# Autodesk Inventor assembly: Space Crush
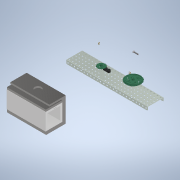
[picture p0: Inventor's stored thumbnail of the model, 180x180]
Saved by Autodesk Inventor 2021 (Build 250183000, 183)
## iProperties
Created: 2021-03-08
Part Number: Space Crush
Document SubType Name: Assembly
Designer: david
Author: david
## Documents named in this file (10)
- C:\Users\david\OneDrive\Documents\Inventor\Space Crush.iam
- C:\Users\david\OneDrive\Documents\Inventor\Inventor_2013_VEX_KOP_-_Imperial\Imperial\Motion\48 Tooth Sprocket.ipt
- C:\Users\david\OneDrive\Documents\Inventor\Inventor_2013_VEX_KOP_-_Imperial\Imperial\Motion\24 Tooth Sprocket.ipt
- C:\Users\david\OneDrive\Documents\Inventor\Inventor_2013_VEX_KOP_-_Imperial\Imperial\Motion\Chain Link.ipt
- C:\Users\david\OneDrive\Documents\Inventor\Inventor_2013_VEX_KOP_-_Imperial\Imperial\Structure\Screw 8-32  x 0.75 inch long.ipt
- C:\Users\david\OneDrive\Documents\Inventor\Inventor_2013_VEX_KOP_-_Imperial\Imperial\Structure\C-Channel 1x5x1x25 Hole.ipt
- C:\Users\david\OneDrive\Documents\Inventor\Inventor_2013_VEX_KOP_-_Imperial\Imperial\Motion\Shaft 2 inch.ipt
- C:\Users\david\OneDrive\Documents\Inventor\Inventor_2013_VEX_KOP_-_Imperial\Imperial\Motion\Bearing Flat.ipt
- C:\Users\david\OneDrive\Documents\Inventor\Clamp for Box Crusher.ipt
- C:\Users\david\OneDrive\Documents\Inventor\Aluminum box 2x2x6 .3 thickness.ipt
## Components (12 placed, 9 different names)
1. 48 Tooth Sprocket:1 — Mate:2, Insert:2, Mate:5
2. 24 Tooth Sprocket:1 — Mate:1, Insert:1, Mate:3
3. Chain Link:1 — Mate:1
4. Chain Link:2 — Mate:2
5. Hexagon Socket Button Head Cap Screw - Inch 8 - 32 x 3/4:1
6. C-Channel 1x5x1x25 Hole:1 — Flush:1, Flush:2, Mate:4, Mate:7
7. Shaft 2 inch:1 — Insert:1, Flush:1, Flush:2
8. Shaft 2 inch:2 — Insert:2, Mate:6
9. Bearing Flat:1 — Mate:3, Mate:4
10. Bearing Flat:2 — Mate:5, Mate:6, Mate:7
11. Clamp for Box Crusher:1 — Mate:8, Flush:3, Mate:9
12. Aluminum box 2x2x6 .3 thickness:1 — Mate:8, Flush:3, Mate:9
## Relationships (14: Mate 9, Flush 3, Insert 2)
- Mate:1: 24 Tooth Sprocket:1 ↔ Chain Link:1
- Mate:2: 48 Tooth Sprocket:1 ↔ Chain Link:2
- Insert:1 (-5.08 mm): 24 Tooth Sprocket:1 ↔ Shaft 2 inch:1
- Flush:1: C-Channel 1x5x1x25 Hole:1 ↔ Shaft 2 inch:1
- Flush:2: C-Channel 1x5x1x25 Hole:1 ↔ Shaft 2 inch:1
- Mate:3: 24 Tooth Sprocket:1 ↔ Bearing Flat:1
- Mate:4: C-Channel 1x5x1x25 Hole:1 ↔ Bearing Flat:1
- Insert:2: 48 Tooth Sprocket:1 ↔ Shaft 2 inch:2
- Mate:5: 48 Tooth Sprocket:1 ↔ Bearing Flat:2
- Mate:6: Shaft 2 inch:2 ↔ Bearing Flat:2
- Mate:7: C-Channel 1x5x1x25 Hole:1 ↔ Bearing Flat:2
- Mate:8: Clamp for Box Crusher:1 ↔ Aluminum box 2x2x6 .3 thickness:1
- Flush:3: Clamp for Box Crusher:1 ↔ Aluminum box 2x2x6 .3 thickness:1
- Mate:9: Clamp for Box Crusher:1 ↔ Aluminum box 2x2x6 .3 thickness:1
